# Autodesk Inventor assembly: bed
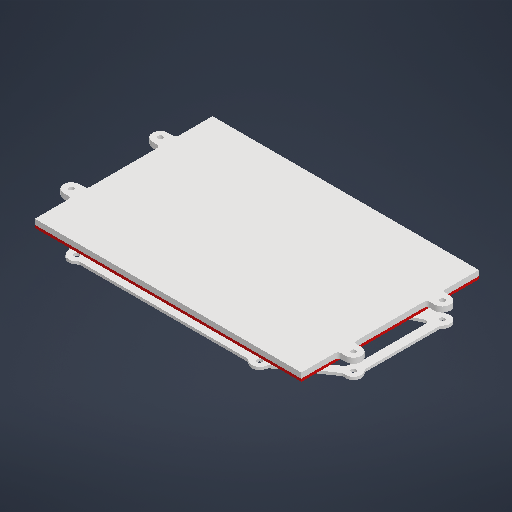
[picture p0: Inventor's stored thumbnail of the model, 512x512]
Saved by Autodesk Inventor 2025 (Build 290162000, 162)
## iProperties
Created: 2024-07-18
Part Number: bed
Document SubType Name: Assembly
Designer: Windows 7 was better
Author: Windows 7 was better
## Documents named in this file (4)
- C:\Users\Windows 7 was better\Documents\GitHub\ReplicatorPlusConversion\CAD\bed.iam
- C:\Users\Windows 7 was better\Documents\GitHub\ReplicatorPlusConversion\CAD\bed-heater.ipt
- C:\Users\Windows 7 was better\Documents\GitHub\ReplicatorPlusConversion\CAD\bed-plate.ipt
- C:\Users\Windows 7 was better\Documents\GitHub\ReplicatorPlusConversion\CAD\bed-interface.ipt
## Components (3 placed, 3 different names)
1. bed-heater:1 — Flush:1
2. bed-plate:1 — Flush:1
3. bed-interface:1
## Relationships (1: Flush 1)
- Flush:1: bed-heater:1 ↔ bed-plate:1
